# Autodesk Inventor assembly: Мостики
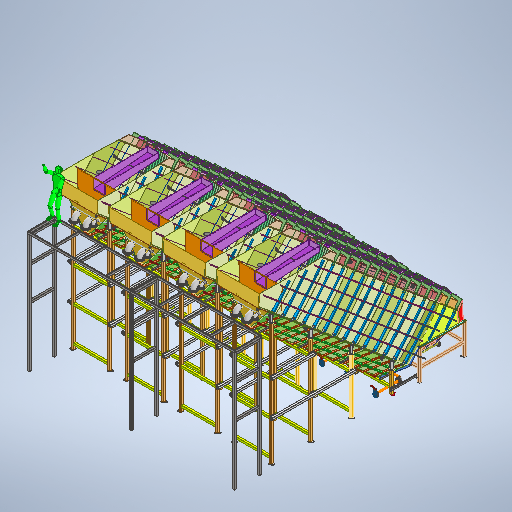
[picture p0: Inventor's stored thumbnail of the model, 512x512]
Saved by Autodesk Inventor 2025 (Build 290162010, 162A)
## iProperties
Created: 2025-01-27
Part Number: Мостики
Document SubType Name: Assembly
Designer: admin
Author: admin
## Documents named in this file (7)
- C:\Users\pokla\Documents\Inventor\Отстойник осветлитель\Manturovo_Se-clar-Gleb\Мостики.iam
- C:\Users\pokla\Documents\Inventor\Отстойник осветлитель\Manturovo_Se-clar-Gleb\ASY MSC 002 отстойник осветлитель.iam
- C:\Users\pokla\Documents\Inventor\Отстойник осветлитель\Manturovo_Se-clar-Gleb\human 01\ч ASY human dummy 01.iam
- C:\Users\pokla\Documents\Inventor\Отстойник осветлитель\Manturovo_Se-clar-Gleb\ASY MSC Платформа отстойников.iam
- C:\Users\pokla\Documents\Inventor\Отстойник осветлитель\Manturovo_Se-clar-Gleb\ASY MSC Опора №1 платф. отст..iam
- C:\Users\pokla\Documents\Inventor\Отстойник осветлитель\Manturovo_Se-clar-Gleb\ASY MSC Опора №2 платф. отст..iam
- C:\Users\pokla\Documents\Inventor\Отстойник осветлитель\Manturovo_Se-clar-Gleb\Габаритные емкости для Димы\Отстойник промывных вод.ipt
## Components (12 placed, 6 different names)
1. ASY MSC 002 отстойник осветлитель:1 [sub-assembly] — Flush:1, Flush:2, Flush:3, Flush:4, Rigid:1, Flush:7, Mate:6
2. ASY MSC 002 отстойник осветлитель:2 [sub-assembly] — Rigid:1, Rigid:2
3. ASY MSC 002 отстойник осветлитель:3 [sub-assembly] — Rigid:3
4. ASY MSC 002 отстойник осветлитель:4 [sub-assembly] — Rigid:2, Rigid:3
5. ч ASY human dummy 01:1 [sub-assembly] — Flush:1
6. ASY MSC Платформа отстойников:1 [sub-assembly] — Rigid:4, Flush:5, Flush:6, Mate:4, Flush:7, Mate:6
7. ASY MSC Опора №1 платф. отст.:1 [sub-assembly] — Flush:5, Flush:6, Mate:4, Rigid:5, Mate:5
8. ASY MSC Опора №1 платф. отст.:2 [sub-assembly] — Rigid:6
9. ASY MSC Опора №2 платф. отст.:1 [sub-assembly]
10. ASY MSC Опора №1 платф. отст.:3 [sub-assembly] — Rigid:5, Rigid:6
11. Отстойник промывных вод:1 — Mate:3
12. ASY MSC Платформа отстойников:2 [sub-assembly] — Rigid:4
## Relationships (17: Flush 7, WeldJoint 6, Mate 4)
- Flush:1 (4500 mm): ASY MSC 002 отстойник осветлитель:1 ↔ ч ASY human dummy 01:1
- Flush:2: ASY MSC 002 отстойник осветлитель:1
- Flush:3: ASY MSC 002 отстойник осветлитель:1
- Flush:4: ASY MSC 002 отстойник осветлитель:1
- Rigid:1 [WeldJoint] (300 mm): ASY MSC 002 отстойник осветлитель:1 ↔ ASY MSC 002 отстойник осветлитель:2
- Rigid:2 [WeldJoint] (300 mm): ASY MSC 002 отстойник осветлитель:2 ↔ ASY MSC 002 отстойник осветлитель:4
- Rigid:3 [WeldJoint] (300 mm): ASY MSC 002 отстойник осветлитель:3 ↔ ASY MSC 002 отстойник осветлитель:4
- Mate:3: Отстойник промывных вод:1
- Rigid:4 [WeldJoint]: ASY MSC Платформа отстойников:1 ↔ ASY MSC Платформа отстойников:2
- Flush:5: ASY MSC Платформа отстойников:1 ↔ ASY MSC Опора №1 платф. отст.:1
- Flush:6: ASY MSC Платформа отстойников:1 ↔ ASY MSC Опора №1 платф. отст.:1
- Mate:4: ASY MSC Платформа отстойников:1 ↔ ASY MSC Опора №1 платф. отст.:1
- Rigid:5 [WeldJoint] (3730 mm): ASY MSC Опора №1 платф. отст.:1 ↔ ASY MSC Опора №1 платф. отст.:3
- Rigid:6 [WeldJoint] (3730 mm): ASY MSC Опора №1 платф. отст.:2 ↔ ASY MSC Опора №1 платф. отст.:3
- Flush:7: ASY MSC 002 отстойник осветлитель:1 ↔ ASY MSC Платформа отстойников:1
- Mate:5: ASY MSC Опора №1 платф. отст.:1
- Mate:6 (500 mm): ASY MSC 002 отстойник осветлитель:1 ↔ ASY MSC Платформа отстойников:1
